# Autodesk Inventor assembly: Rear_Upper_Arm_V1
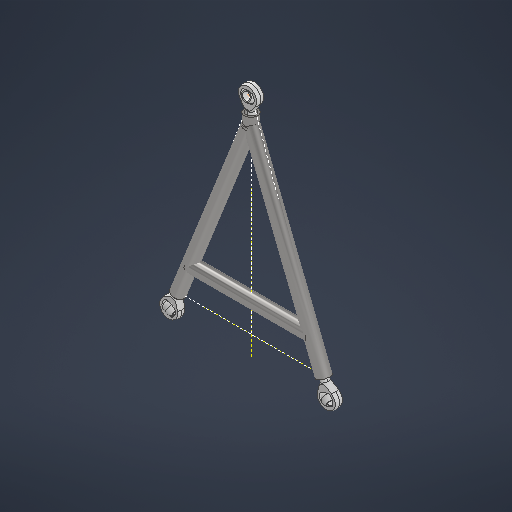
[picture p0: Inventor's stored thumbnail of the model, 512x512]
Saved by Autodesk Inventor 2026.1 (Build 301233000, 233)
## iProperties
Created: 2026-07-13
Part Number: Rear_Upper_Arm_V1
Document SubType Name: Assembly
Designer: share
_SolveAssemblyDoc: Frame Generator Solve Assembly
_Version: 15.0.0
Author: share
## Documents named in this file (4)
- C:\Users\share\OneDrive\Documents\Personal Projects\GOGO Kart\CAD\GOGO_KART_FSAE\Suspension\Suspension Arms\Rear_Upper_Arm_V1\Rear_Upper_Arm_V1.iam
- C:\Users\share\OneDrive\Documents\Personal Projects\GOGO Kart\CAD\GOGO_KART_FSAE\Suspension\Suspension Arms\Arm_Outline_Sketch.ipt
- C:\Users\share\OneDrive\Documents\Personal Projects\GOGO Kart\CAD\GOGO_KART_FSAE\Suspension\Suspension Arms\Rear_Upper_Arm_V1\Rear_Upper_Arm_V1_ Frame.iam
- C:\Users\share\OneDrive\Documents\Personal Projects\GOGO Kart\CAD\GOGO_KART_FSAE\Suspension\Suspension Arms\Suspension Rod Ends\5-8 Rod End Assembly.iam
## Components (5 placed, 3 different names)
1. Arm_Outline_Sketch:1 — Flush:1, Flush:2, Flush:3, Mate:1, Mate:2, Mate:4, Mate:5, Mate:7, Mate:9
2. Rear_Upper_Arm_V1_ Frame:1 [sub-assembly]
3. 5-8 Rod End Assembly:1 [sub-assembly] — Mate:1, Mate:2, Mate:3
4. 5-8 Rod End Assembly:2 [sub-assembly] — Mate:4, Mate:5, Mate:6
5. 5-8 Rod End Assembly:3 [sub-assembly] — Mate:7, Mate:8, Mate:9
## Relationships (12: Mate 9, Flush 3)
- Flush:1: Arm_Outline_Sketch:1
- Flush:2: Arm_Outline_Sketch:1
- Flush:3: Arm_Outline_Sketch:1
- Mate:1: Arm_Outline_Sketch:1 ↔ 5-8 Rod End Assembly:1
- Mate:2: Arm_Outline_Sketch:1 ↔ 5-8 Rod End Assembly:1
- Mate:3: 5-8 Rod End Assembly:1
- Mate:4: Arm_Outline_Sketch:1 ↔ 5-8 Rod End Assembly:2
- Mate:5: Arm_Outline_Sketch:1 ↔ 5-8 Rod End Assembly:2
- Mate:6: 5-8 Rod End Assembly:2
- Mate:7: Arm_Outline_Sketch:1 ↔ 5-8 Rod End Assembly:3
- Mate:8: 5-8 Rod End Assembly:3
- Mate:9: Arm_Outline_Sketch:1 ↔ 5-8 Rod End Assembly:3
